# Autodesk Inventor assembly: Rotor
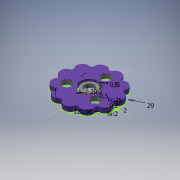
[picture p0: Inventor's stored thumbnail of the model, 180x180]
Saved by Autodesk Inventor 2018.3 (Build 223284000, 284)
## iProperties
Created: 2018-08-03
Part Number: Rotor
Material: Generisch
Document SubType Name: Assembly
Designer: JochenAlt
Author: JochenAlt
## Documents named in this file (4)
- D:\Projects\FlowerPot\CAD\CycloidalGear2\Rotor.iam
- D:\Projects\FlowerPot\CAD\CycloidalGear2\Rotor.ipt
- Excenter1.ipt
- D:\Projects\FlowerPot\CAD\CycloidalGear\W 61700 X-2RS1.iam
## Components (5 placed, 2 different names)
1. Excenter1:1 — Passend:1, Passend:2, Passend:3, Passend:4, Fluchtend:1, Fluchtend:2, Fluchtend:3, Fluchtend:4
2. W 61700 X-2RS1:1 [sub-assembly] — Passend:1, Fluchtend:1
3. W 61700 X-2RS1:2 [sub-assembly] — Passend:3, Fluchtend:4
4. W 61700 X-2RS1:3 [sub-assembly] — Passend:2, Fluchtend:2
5. W 61700 X-2RS1:4 [sub-assembly] — Passend:4, Fluchtend:3
## Relationships (8: Mate 4, Flush 4)
- Passend:1 [Mate]: Excenter1:1 ↔ W 61700 X-2RS1:1
- Passend:2 [Mate]: Excenter1:1 ↔ W 61700 X-2RS1:3
- Passend:3 [Mate]: Excenter1:1 ↔ W 61700 X-2RS1:2
- Passend:4 [Mate]: Excenter1:1 ↔ W 61700 X-2RS1:4
- Fluchtend:1 [Flush] (0.5 mm): Excenter1:1 ↔ W 61700 X-2RS1:1
- Fluchtend:2 [Flush] (0.5 mm): Excenter1:1 ↔ W 61700 X-2RS1:3
- Fluchtend:3 [Flush] (0.5 mm): Excenter1:1 ↔ W 61700 X-2RS1:4
- Fluchtend:4 [Flush] (0.5 mm): Excenter1:1 ↔ W 61700 X-2RS1:2
